# Autodesk Inventor assembly: Estructura_bk
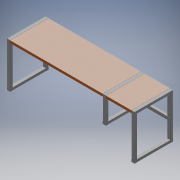
[picture p0: Inventor's stored thumbnail of the model, 180x180]
Saved by Autodesk Inventor 2016 (Build 200138000, 138)
## iProperties
Created: 2018-06-24
Part Number: Estructura_bk
Document SubType Name: Assembly
Designer: damia
_SolveAssemblyDoc: Frame Generator Solve Assembly
_Version: 15.0.0
Author: damia
## Documents named in this file (5)
- C:\Users\damia\Documents\Inventor\escritorio_Damian\Estructura_bk.iam
- C:\Users\damia\Documents\Inventor\Escritorio_Damian\Esqueleto.ipt
- C:\Users\damia\Documents\Inventor\Escritorio_Damian\Estructura\Frame\Frame0002.iam
- C:\Users\damia\Documents\Inventor\Escritorio_Damian\Part42.ipt
- C:\Users\damia\Documents\Inventor\Escritorio_Damian\VidrioChico.ipt
## Components (4 placed, 4 different names)
1. Esqueleto:1 — Mate:1, Mate:2
2. Frame0002:1 [sub-assembly] — Flush:1, Flush:2, Flush:3, Flush:4
3. VidrioGrande:1 — Flush:1, Flush:2
4. VidrioChico:1 — Flush:3, Flush:4
## Relationships (6: Flush 4, Mate 2)
- Mate:1: Esqueleto:1
- Mate:2: Esqueleto:1
- Flush:1: Frame0002:1 ↔ VidrioGrande:1
- Flush:2: Frame0002:1 ↔ VidrioGrande:1
- Flush:3: Frame0002:1 ↔ VidrioChico:1
- Flush:4: Frame0002:1 ↔ VidrioChico:1
